# Autodesk Inventor assembly: 15102898-16-A-1000
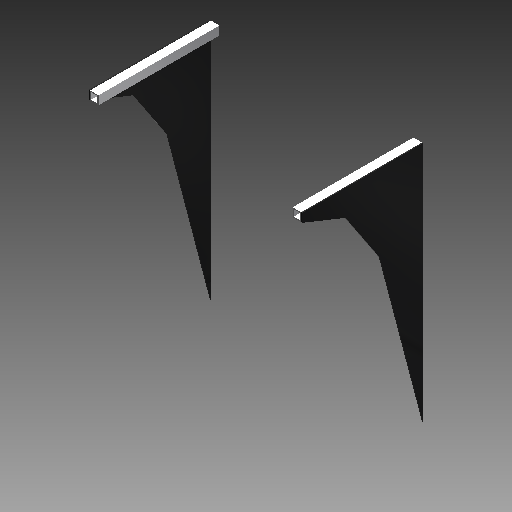
[picture p0: Inventor's stored thumbnail of the model, 512x512]
Saved by Autodesk Inventor 2017 (Build 210142000, 142)
## iProperties
Created: 2016-11-08
Part Number: 15102898-16-A-1000
Document SubType Name: Assembly
Designer: gus
Author: gus
## Documents named in this file (3)
- \\Mac\Home\Desktop\bunnybots 2016\15102898-16-Bunnybot-CAD\Bunnybot-Night_Fury\15102898-16-A-0000\15102898-16-A-1000\15102898-16-A-1000.iam
- \\Mac\Home\Desktop\bunnybots 2016\15102898-16-Bunnybot-CAD\Bunnybot-Night_Fury\15102898-16-A-0000\15102898-16-A-1000\15102898-16-P-0101.ipt
- \\Mac\Home\Desktop\bunnybots 2016\15102898-16-Bunnybot-CAD\Bunnybot-Night_Fury\15102898-16-A-0000\15102898-16-A-1000\15102898-16-P-0102.ipt
## Components (4 placed, 2 different names)
1. 15102898-16-P-0101:1 — Flush:1, Flush:2, Mate:1, Flush:5, Flush:6
2. 15102898-16-P-0102:1 — Flush:1, Flush:2, Mate:1
3. 15102898-16-P-0102:2 — Mate:2, Flush:3, Flush:4
4. 15102898-16-P-0101:2 — Mate:2, Flush:3, Flush:4, Flush:5, Flush:6
## Relationships (8: Flush 6, Mate 2)
- Flush:1: 15102898-16-P-0101:1 ↔ 15102898-16-P-0102:1
- Flush:2: 15102898-16-P-0101:1 ↔ 15102898-16-P-0102:1
- Mate:1: 15102898-16-P-0101:1 ↔ 15102898-16-P-0102:1
- Mate:2: 15102898-16-P-0102:2 ↔ 15102898-16-P-0101:2
- Flush:3: 15102898-16-P-0102:2 ↔ 15102898-16-P-0101:2
- Flush:4: 15102898-16-P-0102:2 ↔ 15102898-16-P-0101:2
- Flush:5: 15102898-16-P-0101:1 ↔ 15102898-16-P-0101:2
- Flush:6: 15102898-16-P-0101:1 ↔ 15102898-16-P-0101:2
